# Autodesk Inventor assembly: Chappie
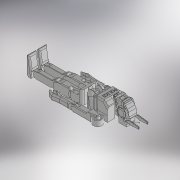
[picture p0: Inventor's stored thumbnail of the model, 180x180]
Saved by Autodesk Inventor 2022 (Build 260153000, 153)
## iProperties
Created: 2022-02-25
Part Number: Chappie
Document SubType Name: Assembly
Designer: joshw
Author: joshw
## Documents named in this file (11)
- C:\Users\joshw\Desktop\fun\Assembly\Chappie.iam
- C:\Users\joshw\Desktop\fun\Part\Body.ipt
- C:\Users\joshw\Desktop\fun\Part\Head.ipt
- C:\Users\joshw\Desktop\fun\Part\Sholder.ipt
- C:\Users\joshw\Desktop\fun\Part\Upper Arm.ipt
- C:\Users\joshw\Desktop\fun\Part\lOWER ARM.ipt
- C:\Users\joshw\Desktop\fun\Part\hIP.ipt
- C:\Users\joshw\Desktop\fun\Part\Upper Leg.ipt
- C:\Users\joshw\Desktop\fun\Part\Lower Leg.ipt
- C:\Users\joshw\Desktop\fun\Part\Foot.ipt
- C:\Users\joshw\Desktop\fun\Part\Upper Leg_oposite.ipt
## Components (15 placed, 10 different names)
1. Body:1 — Mate:1, Mate:2, Angle:1, Mate:3, Mate:4, Mate:5, Angle:2, Flush:1, Angle:3, Mate:14, Angle:6, Mate:15, Angle:12, Mate:34, Mate:35, Angle:14, Angle:16
2. Head:1 — Mate:2, Angle:1, Mate:3, Flush:2, Flush:6
3. Sholder:1 — Mate:4, Mate:5, Mate:6, Angle:2
4. Upper Arm:1 — Mate:6, Flush:1, Angle:3, Mate:8, Mate:9, Flush:3
5. lOWER ARM:1 — Mate:8, Mate:9, Flush:3
6. hIP:1 — Mate:14, Angle:6, Mate:15, Mate:16, Mate:17, Angle:7, Mate:27, Mate:30
7. Upper Leg:1 — Mate:16, Mate:17, Angle:7, Mate:18, Mate:19, Angle:8
8. Lower Leg:1 — Mate:18, Mate:19, Angle:8, Mate:20, Mate:21, Angle:9
9. Foot:1 — Mate:20, Mate:21, Angle:9
10. Lower Leg:2 — Mate:28, Mate:29, Angle:13
11. Foot:2
12. Upper Leg_oposite:1 — Mate:27, Mate:28, Mate:29, Mate:30, Angle:12, Angle:13
13. Sholder:2 — Flush:8, Mate:34, Mate:35, Angle:16
14. Upper Arm:2 — Mate:32, Mate:33, Flush:8, Angle:14, Angle:15
15. lOWER ARM:2 — Mate:32, Mate:33, Angle:15
## Relationships (45: Mate 27, Angle 13, Flush 5)
- Mate:1: Body:1
- Mate:2 (0.45 mm): Body:1 ↔ Head:1
- Angle:1 (0 deg): Body:1 ↔ Head:1
- Mate:3: Body:1 ↔ Head:1
- Mate:4: Body:1 ↔ Sholder:1
- Mate:5 (0.75 mm): Body:1 ↔ Sholder:1
- Mate:6: Sholder:1 ↔ Upper Arm:1
- Angle:2 (0 deg): Body:1 ↔ Sholder:1
- Flush:1: Body:1 ↔ Upper Arm:1
- Angle:3 (0 deg): Body:1 ↔ Upper Arm:1
- Flush:2: Head:1
- Mate:8: Upper Arm:1 ↔ lOWER ARM:1
- Mate:9 (0.375 mm): Upper Arm:1 ↔ lOWER ARM:1
- Flush:3: Upper Arm:1 ↔ lOWER ARM:1
- Mate:14: Body:1 ↔ hIP:1
- Angle:6 (0 deg): Body:1 ↔ hIP:1
- Mate:15 (0.5 mm): Body:1 ↔ hIP:1
- Mate:16: hIP:1 ↔ Upper Leg:1
- Mate:17 (0.45 mm): hIP:1 ↔ Upper Leg:1
- Angle:7 (0 deg): hIP:1 ↔ Upper Leg:1
- Mate:18: Upper Leg:1 ↔ Lower Leg:1
- Mate:19 (0.45 mm): Upper Leg:1 ↔ Lower Leg:1
- Angle:8 (0 deg): Upper Leg:1 ↔ Lower Leg:1
- Mate:20: Lower Leg:1 ↔ Foot:1
- Mate:21 (0.45 mm): Lower Leg:1 ↔ Foot:1
- Angle:9 (0 deg): Lower Leg:1 ↔ Foot:1
- [Mate]: Lower Leg:2 ↔ Foot:2
- [Mate] (0.45 mm): Lower Leg:2 ↔ Foot:2
- [Angle] (0 deg): Lower Leg:2 ↔ Foot:2
- Mate:27 (0.45 mm): hIP:1 ↔ Upper Leg_oposite:1
- Mate:28: Lower Leg:2 ↔ Upper Leg_oposite:1
- Mate:29 (0.45 mm): Lower Leg:2 ↔ Upper Leg_oposite:1
- Mate:30: hIP:1 ↔ Upper Leg_oposite:1
- Angle:12 (0 deg): Body:1 ↔ Upper Leg_oposite:1
- Angle:13 (0 deg): Lower Leg:2 ↔ Upper Leg_oposite:1
- Flush:6 (20.75 mm): Head:1
- [Mate]: Sholder:2 ↔ Upper Arm:2
- Mate:32: Upper Arm:2 ↔ lOWER ARM:2
- Mate:33 (0.375 mm): Upper Arm:2 ↔ lOWER ARM:2
- Flush:8: Sholder:2 ↔ Upper Arm:2
- Mate:34: Body:1 ↔ Sholder:2
- Mate:35 (0.75 mm): Body:1 ↔ Sholder:2
- Angle:14 (0 deg): Body:1 ↔ Upper Arm:2
- Angle:15 (0 deg): Upper Arm:2 ↔ lOWER ARM:2
- Angle:16 (0 deg): Body:1 ↔ Sholder:2
## Named parameters: d44_d38 = 0 mm, d45_d39 = 0.45 mm, d46_d40 = 0 deg, d58_d6 = 0 mm, d59_d14 = 0 mm, d60_d15 = 0.375 mm
